# Autodesk Inventor assembly: IMU
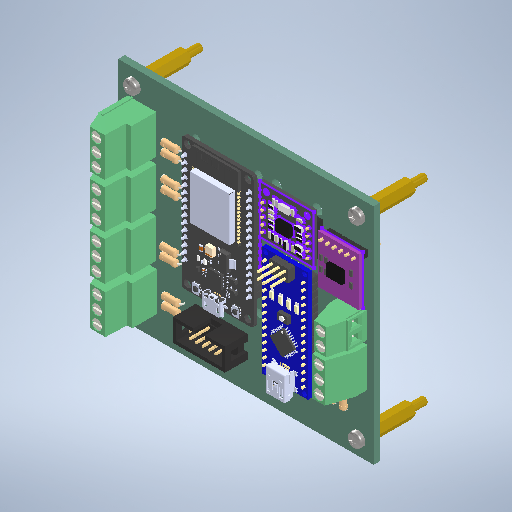
[picture p0: Inventor's stored thumbnail of the model, 512x512]
Saved by Autodesk Inventor 2025.2 (Build 292293000, 293)
## iProperties
Company: Kicad
Created: 2025-02-24
Part Number: IMU
Description: KiCad electronic assembly
Document SubType Name: Assembly
Designer: nugro
Authority: Unknown
Sending System: KiCad to STEP converter
Preprocessor: Open CASCADE STEP processor 7.8
Title: IMU.step
Author: Pcbnew
## Documents named in this file (4)
- C:\Users\nugro\Documents\KiCad\IMU\IMU\IMU\IMU.iam
- C:\Users\nugro\Downloads\m3-standoff-pcb-spacers-1.snapshot.2\M3_M_TO_F_20MM_STANDOFF\M3_M_TO_F_20MM_STANDOFF\M3_M_TO_F_20MM_STANDOFF.ipt
- C:\Users\nugro\Documents\Inventor\Content Center Files\R2025\en-US\JIS B 1111  Z (2)\JIS B 1111 - A M3 x 4 - Z(1).ipt
- C:\Users\nugro\Documents\KiCad\IMU\IMU\IMU\IMU.ipt
## Components (9 placed, 3 different names)
1. M3_M_TO_F_20MM_STANDOFF:1 — Mate:6
2. M3_M_TO_F_20MM_STANDOFF:2 — Mate:7
3. M3_M_TO_F_20MM_STANDOFF:3 — Insert:1
4. M3_M_TO_F_20MM_STANDOFF:4 — Mate:5
5. JIS B 1111 Z - Metric A M3 x 4 - Z:1 — Insert:1, Mate:11
6. JIS B 1111 Z - Metric A M3 x 4 - Z:2 — Mate:5, Mate:10
7. JIS B 1111 Z - Metric A M3 x 4 - Z:3 — Mate:6, Mate:9
8. JIS B 1111 Z - Metric A M3 x 4 - Z:4 — Mate:7, Mate:8
9. IMU:1 — Mate:8, Mate:9, Mate:10, Mate:11
## Relationships (8: Mate 7, Insert 1)
- Insert:1: M3_M_TO_F_20MM_STANDOFF:3 ↔ JIS B 1111 Z - Metric A M3 x 4 - Z:1
- Mate:5: M3_M_TO_F_20MM_STANDOFF:4 ↔ JIS B 1111 Z - Metric A M3 x 4 - Z:2
- Mate:6: M3_M_TO_F_20MM_STANDOFF:1 ↔ JIS B 1111 Z - Metric A M3 x 4 - Z:3
- Mate:7: M3_M_TO_F_20MM_STANDOFF:2 ↔ JIS B 1111 Z - Metric A M3 x 4 - Z:4
- Mate:8: JIS B 1111 Z - Metric A M3 x 4 - Z:4 ↔ IMU:1
- Mate:9: JIS B 1111 Z - Metric A M3 x 4 - Z:3 ↔ IMU:1
- Mate:10: JIS B 1111 Z - Metric A M3 x 4 - Z:2 ↔ IMU:1
- Mate:11: JIS B 1111 Z - Metric A M3 x 4 - Z:1 ↔ IMU:1
